# Autodesk Inventor assembly: 502.001.01_Linearaktor
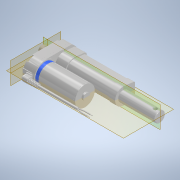
[picture p0: Inventor's stored thumbnail of the model, 180x180]
Saved by Autodesk Inventor 2022 (Build 260153000, 153)
## iProperties
Created: 2021-11-14
Part Number: 502.001.01_Linearaktor
Document SubType Name: Assembly
Designer: Oliver Ungerer
KODE_ZEICHNUNGSNUMMER: CAHB-10-B1A-050158-AAAA0A-000
BENENNUNG: -
MASSE: 0.760195
PDMREV: 0.0+
PDMRL: Entwicklung
PROI_REVISION: 0
PROI_VERSION: 0+
PROI_RELEASE: Entwicklung
PTC_MODIFIED: True
PROI_CREATED_BY: Kantioler_adm
PROI_CREATED_ON: 07.03.2008 12:11:19
PROI_LOCATION: Root-Ordner/Pro_stds/Start_Files
MATERIALART: -
EINHEIT: ST
HERSTELLER_PREIS: 0.0
PTC_ORGANIZATION_ID: Durst
PTC_WM_REVISION: 0
PTC_WM_ITERATION: 0
PTC_WM_VERSION: 0.0
PTC_WM_LIFECYCLE_STATE: Entwicklung
PTC_WM_LIFECYCLE: 02 Durst
PTC_WM_CREATED_BY: Oliver Ungerer (oungerer: Durst)
PTC_WM_CREATED_ON: 01.08.21
PTC_WM_MODIFIED_BY: Oliver Ungerer (oungerer: Durst)
PTC_WM_MODIFIED_ON: 01.08.21
AEND_INDEX: 0
VERSION: 0
STATUS: 0.0
PTC_VAL_IMP_SCORE: PASS
Author: Oliver Ungerer
## Documents named in this file (3)
- C:\Users\kaebi\OneDrive - mci4me.at\03_MCI Master\4.Semester_SS2022\Masterarbeit\Software\CAD_TeachingFactory\506.007.01_Linearaktor.iam
- C:\Users\kaebi\OneDrive - mci4me.at\03_MCI Master\4.Semester_SS2022\Masterarbeit\Software\CAD_TeachingFactory\506.006.01_CAHB10-050-AA-0-A-B.ipt
- C:\Users\kaebi\OneDrive - mci4me.at\03_MCI Master\4.Semester_SS2022\Masterarbeit\Software\CAD_TeachingFactory\506.005.01_CAHB10-050-0-AA-A-R.ipt
## Components (2 placed, 2 different names)
1. 506.006.01_CAHB10-050-AA-0-A-B — Passend:1
2. 506.005.01_CAHB10-050-0-AA-A-R — Passend:1
## Relationships (1: Mate 1)
- Passend:1 [Mate]: 506.006.01_CAHB10-050-AA-0-A-B ↔ 506.005.01_CAHB10-050-0-AA-A-R
